# Autodesk Inventor assembly: boat_assm_2
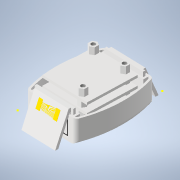
[picture p0: Inventor's stored thumbnail of the model, 180x180]
Saved by Autodesk Inventor 2020 (Build 240168000, 168)
## iProperties
Created: 2020-05-14
Part Number: boat_assm_2
Document SubType Name: Assembly
Designer: nicva
Author: nicva
## Documents named in this file (6)
- C:\Users\nicva\Documents\Microbots\Boat\Inventor\boat_assm_2.iam
- C:\Users\nicva\Documents\Microbots\Boat\Inventor\NVO_boat5.ipt
- C:\Users\nicva\Documents\Microbots\Boat\Inventor\IDT_Mount_23_3.ipt
- C:\Users\nicva\Documents\Microbots\Boat\Inventor\Standoff_screw_model_2.ipt
- C:\Users\nicva\Documents\Microbots\Boat\Inventor\PCB_model_2.ipt
- C:\Users\nicva\Documents\Microbots\Boat\Inventor\Device21.ipt
## Components (17 placed, 5 different names)
1. NVO_boat5:1 — Slider:1, Slider:2, Mate:1, Mate:2, Cylindrical:1, Cylindrical:2, Cylindrical:3
2. IDT_Mount_23_3:1 — Slider:2, Slider:4
3. IDT_Mount_23_3:2 — Slider:1, Slider:3
4. Standoff_screw_model_2:1 — Cylindrical:7
5. Standoff_screw_model_2:2 — Cylindrical:5, Cylindrical:9
6. Standoff_screw_model_2:4 — Cylindrical:9
7. Standoff_screw_model_2:6 — Cylindrical:8
8. Standoff_screw_model_2:8 — Cylindrical:6, Mate:5, Cylindrical:8
9. Standoff_screw_model_2:9 — Cylindrical:4, Mate:6, Cylindrical:7
10. Standoff_screw_model_2:10 — Cylindrical:1, Mate:3, Cylindrical:4
11. Standoff_screw_model_2:11 — Cylindrical:3, Mate:4, Cylindrical:6
12. Standoff_screw_model_2:12 — Cylindrical:2, Cylindrical:5
13. PCB_model_2:1 — Mate:1, Mate:2
14. PCB_model_2:2 — Mate:3, Mate:4
15. PCB_model_2:3 — Mate:5, Mate:6
16. Device21:1 — Slider:3
17. Device21:2 — Slider:4
## Relationships (19: CylindricalJoint 9, Mate 6, TranslationJoint 4)
- Slider:1 [TranslationJoint]: NVO_boat5:1 ↔ IDT_Mount_23_3:2
- Slider:2 [TranslationJoint]: NVO_boat5:1 ↔ IDT_Mount_23_3:1
- Mate:1: NVO_boat5:1 ↔ PCB_model_2:1
- Mate:2: NVO_boat5:1 ↔ PCB_model_2:1
- Cylindrical:1: NVO_boat5:1 ↔ Standoff_screw_model_2:10
- Cylindrical:2: NVO_boat5:1 ↔ Standoff_screw_model_2:12
- Cylindrical:3: NVO_boat5:1 ↔ Standoff_screw_model_2:11
- Mate:3: Standoff_screw_model_2:10 ↔ PCB_model_2:2
- Mate:4: Standoff_screw_model_2:11 ↔ PCB_model_2:2
- Cylindrical:4: Standoff_screw_model_2:9 ↔ Standoff_screw_model_2:10
- Cylindrical:5: Standoff_screw_model_2:2 ↔ Standoff_screw_model_2:12
- Cylindrical:6: Standoff_screw_model_2:8 ↔ Standoff_screw_model_2:11
- Mate:5: Standoff_screw_model_2:8 ↔ PCB_model_2:3
- Mate:6: Standoff_screw_model_2:9 ↔ PCB_model_2:3
- Cylindrical:7: Standoff_screw_model_2:1 ↔ Standoff_screw_model_2:9
- Cylindrical:8: Standoff_screw_model_2:6 ↔ Standoff_screw_model_2:8
- Cylindrical:9: Standoff_screw_model_2:2 ↔ Standoff_screw_model_2:4
- Slider:3 [TranslationJoint]: IDT_Mount_23_3:2 ↔ Device21:1
- Slider:4 [TranslationJoint]: IDT_Mount_23_3:1 ↔ Device21:2
